# Autodesk Inventor assembly: Assembly1
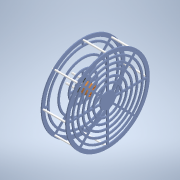
[picture p0: Inventor's stored thumbnail of the model, 180x180]
Saved by Autodesk Inventor 2021 (Build 250183000, 183)
## iProperties
Created: 2023-10-20
Part Number: Assembly1
Document SubType Name: Assembly
Designer: Lenovo
Mass: 216.424 g
Surface Area: 1443.24 cm^2
Volume: 135.689 cm^3
Density: 1.59499 g/cm^3
Author: Lenovo
## Documents named in this file (7)
- E:\0 semester 10\GP2\2DOF_Hover\CAD\Workspaces\Workspace\Assembly1.iam
- E:\0 semester 10\GP2\2DOF_Hover\CAD\Workspaces\Workspace\Part1.ipt
- E:\0 semester 10\GP2\2DOF_Hover\CAD\Workspaces\Workspace\Part16.ipt
- E:\0 semester 10\GP2\2DOF_Hover\CAD\Workspaces\Workspace\Part17.ipt
- E:\0 semester 10\GP2\2DOF_Hover\CAD\Workspaces\Workspace\Part18.ipt
- E:\0 semester 10\GP2\2DOF_Hover\CAD\Workspaces\Workspace\spacers for prop.ipt
- E:\0 semester 10\GP2\2DOF_Hover\CAD\Workspaces\Workspace\Standoff M3 M-M H 45mm.ipt
## Components (16 placed, 6 different names)
1. Part1:1 — Mate:25, Mate:26, Mate:27
2. Part16:1 — Mate:10, Mate:11, Mate:12, Mate:29, Mate:31, Mate:33, Mate:34, Mate:35, Mate:37, Mate:38, Mate:39, Mate:40, Mate:41, Mate:42, Mate:43
3. Part17:1 — Mate:10, Mate:11, Mate:12, Mate:21, Mate:22, Mate:23, Mate:24, Mate:28, Mate:30, Mate:32, Mate:36, Mate:44, Mate:45, Mate:46, Mate:47, Mate:48, Mate:49, Mate:50, Mate:51
4. Part18:1 — Mate:22, Mate:23, Mate:24, Mate:25, Mate:26, Mate:27
5. spacers for prop:1 — Mate:28, Mate:29
6. spacers for prop:2 — Mate:30, Mate:31
7. spacers for prop:3 — Mate:32, Mate:33
8. spacers for prop:4 — Mate:34, Mate:35
9. spacers for prop:5 — Mate:36, Mate:37
10. spacers for prop:6 — Mate:40, Mate:41
11. spacers for prop:7 — Mate:42, Mate:43
12. spacers for prop:8 — Mate:38, Mate:39
13. Standoff M3 M-M H 45mm:1 — Mate:44, Mate:45
14. Standoff M3 M-M H 45mm:2 — Mate:46, Mate:47
15. Standoff M3 M-M H 45mm:3 — Mate:48, Mate:49
16. Standoff M3 M-M H 45mm:4 — Mate:50, Mate:51
## Relationships (34: Mate 34)
- Mate:10: Part16:1 ↔ Part17:1
- Mate:11: Part16:1 ↔ Part17:1
- Mate:12 (67 mm): Part16:1 ↔ Part17:1
- Mate:21: Part17:1
- Mate:22: Part17:1 ↔ Part18:1
- Mate:23: Part17:1 ↔ Part18:1
- Mate:24: Part17:1 ↔ Part18:1
- Mate:25: Part1:1 ↔ Part18:1
- Mate:26: Part1:1 ↔ Part18:1
- Mate:27: Part1:1 ↔ Part18:1
- Mate:28: Part17:1 ↔ spacers for prop:1
- Mate:29: Part16:1 ↔ spacers for prop:1
- Mate:30: Part17:1 ↔ spacers for prop:2
- Mate:31: Part16:1 ↔ spacers for prop:2
- Mate:32: Part17:1 ↔ spacers for prop:3
- Mate:33: Part16:1 ↔ spacers for prop:3
- Mate:34: Part16:1 ↔ spacers for prop:4
- Mate:35: Part16:1 ↔ spacers for prop:4
- Mate:36: Part17:1 ↔ spacers for prop:5
- Mate:37: Part16:1 ↔ spacers for prop:5
- Mate:38: Part16:1 ↔ spacers for prop:8
- Mate:39: Part16:1 ↔ spacers for prop:8
- Mate:40: Part16:1 ↔ spacers for prop:6
- Mate:41: Part16:1 ↔ spacers for prop:6
- Mate:42: Part16:1 ↔ spacers for prop:7
- Mate:43: Part16:1 ↔ spacers for prop:7
- Mate:44: Part17:1 ↔ Standoff M3 M-M H 45mm:1
- Mate:45: Part17:1 ↔ Standoff M3 M-M H 45mm:1
- Mate:46: Part17:1 ↔ Standoff M3 M-M H 45mm:2
- Mate:47: Part17:1 ↔ Standoff M3 M-M H 45mm:2
- Mate:48: Part17:1 ↔ Standoff M3 M-M H 45mm:3
- Mate:49: Part17:1 ↔ Standoff M3 M-M H 45mm:3
- Mate:50: Part17:1 ↔ Standoff M3 M-M H 45mm:4
- Mate:51: Part17:1 ↔ Standoff M3 M-M H 45mm:4
